# Autodesk Inventor assembly: 3_disenio_derivado_mas_stock_resina
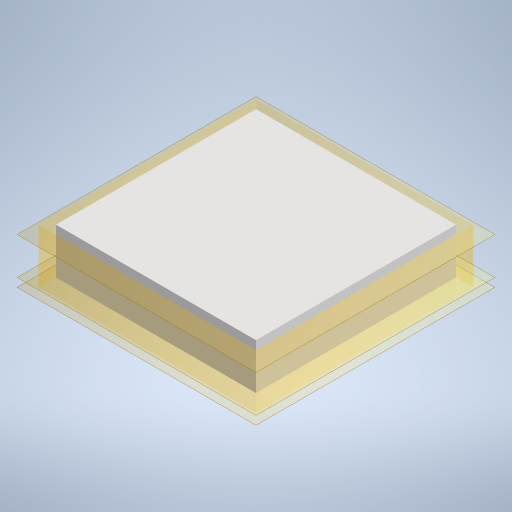
[picture p0: Inventor's stored thumbnail of the model, 512x512]
Saved by Autodesk Inventor 2023.2 (Build 272271030, 271C)
## iProperties
Created: 2023-08-30
Part Number: 3_disenio_derivado_mas_stock_resina
Document SubType Name: Assembly
Designer: Cris Pat
Author: Cris Pat
## Documents named in this file (3)
- C:\Users\Cris Pat\Desktop\U\Semestre_10\Disenio_y_manufactura\Molde_Github\3_disenio_derivado_mas_stock_resina.iam
- C:\Users\Cris Pat\Desktop\U\Semestre_10\Disenio_y_manufactura\Molde_Github\2_disenio_derivado.ipt
- C:\Users\Cris Pat\Desktop\U\Semestre_10\Disenio_y_manufactura\Molde_Github\STOCK_MATERIAL_1.ipt
## Components (2 placed, 2 different names)
1. 2_disenio_derivado:1
2. STOCK_MATERIAL_1:1 — Flush:1
## Relationships (1: Flush 1)
- Flush:1: STOCK_MATERIAL_1:1
